# Autodesk Inventor assembly: KON_Nietmaschine_Dorn
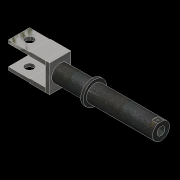
[picture p0: Inventor's stored thumbnail of the model, 180x180]
Saved by Autodesk Inventor 2019 (Build 230136000, 136)
## iProperties
Created: 2021-12-29
Part Number: KON_Nietmaschine_Dorn
Material: Generisch
Document SubType Name: Weldment
Designer: Jonas Nebl
Weld Material: Welded Aluminum-6061
Mass: 1625.74 g
Surface Area: 451.059 cm^2
Volume: 207.123 cm^3
Density: 7.84919 g/cm^3
Author: Jonas Nebl
## Documents named in this file (5)
- C:\Users\jonas\Documents\Inventor\Nietmaschine\KON_Nietmaschine_Dorn.iam
- C:\Users\jonas\Documents\Inventor\Nietmaschine\KON_Nietmaschine_Dorn.ipt
- C:\Users\jonas\Documents\Inventor\Nietmaschine\EN 10058 - 40 x 6 - 46.ipt
- C:\Users\jonas\Documents\Inventor\Nietmaschine\EN 10058 - 40 x 6 - 60.ipt
- C:\Users\jonas\Documents\Inventor\Content Center Files\R2019\de-DE\ISO 4762(1)\DIN EN ISO 4762 - M6 x 16.ipt
## Components (6 placed, 4 different names)
1. KON_Nietmaschine_Dorn:1 — Passend:1, Tangential:1, Tangential:2
2. EN 10058 - 40 x 6 - 46:1 — Passend:1, Passend:2, Passend:3, Fluchtend:1, Fluchtend:2, Fluchtend:3, Fluchtend:4, Tangential:2, Einfügen:1, Einfügen:2
3. EN 10058 - 40 x 6 - 60:1 — Passend:3, Fluchtend:1, Fluchtend:2
4. EN 10058 - 40 x 6 - 60:2 — Passend:2, Fluchtend:3, Fluchtend:4, Tangential:1
5. DIN EN ISO 4762 M6 x 16:1 — Einfügen:1
6. DIN EN ISO 4762 M6 x 16:2 — Einfügen:2
## Relationships (11: Flush 4, Mate 3, Tangent 2, Insert 2)
- Passend:1 [Mate]: KON_Nietmaschine_Dorn:1 ↔ EN 10058 - 40 x 6 - 46:1
- Passend:2 [Mate]: EN 10058 - 40 x 6 - 46:1 ↔ EN 10058 - 40 x 6 - 60:2
- Passend:3 [Mate]: EN 10058 - 40 x 6 - 46:1 ↔ EN 10058 - 40 x 6 - 60:1
- Fluchtend:1 [Flush]: EN 10058 - 40 x 6 - 46:1 ↔ EN 10058 - 40 x 6 - 60:1
- Fluchtend:2 [Flush]: EN 10058 - 40 x 6 - 46:1 ↔ EN 10058 - 40 x 6 - 60:1
- Fluchtend:3 [Flush]: EN 10058 - 40 x 6 - 46:1 ↔ EN 10058 - 40 x 6 - 60:2
- Fluchtend:4 [Flush]: EN 10058 - 40 x 6 - 46:1 ↔ EN 10058 - 40 x 6 - 60:2
- Tangential:1 (4 mm): KON_Nietmaschine_Dorn:1 ↔ EN 10058 - 40 x 6 - 60:2
- Tangential:2 (-2 mm): KON_Nietmaschine_Dorn:1 ↔ EN 10058 - 40 x 6 - 46:1
- Einfügen:1 [Insert]: EN 10058 - 40 x 6 - 46:1 ↔ DIN EN ISO 4762 M6 x 16:1
- Einfügen:2 [Insert]: EN 10058 - 40 x 6 - 46:1 ↔ DIN EN ISO 4762 M6 x 16:2
